# Autodesk Inventor assembly: serwo_v2
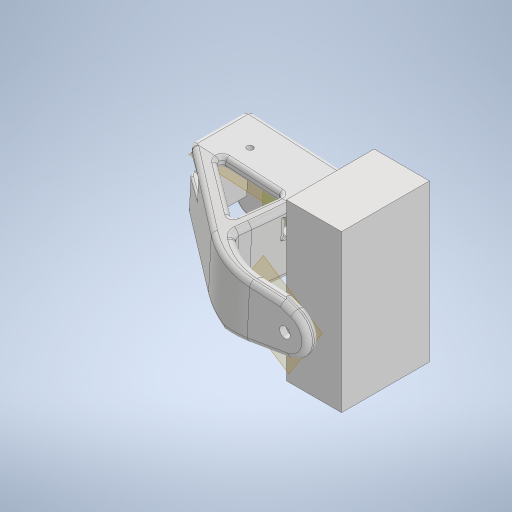
[picture p0: Inventor's stored thumbnail of the model, 512x512]
Saved by Autodesk Inventor 2023 (Build 270158000, 158)
## iProperties
Created: 2024-06-29
Part Number: serwo_v2
Document SubType Name: Assembly
Designer: kamil
Author: kamil
## Documents named in this file (4)
- C:\Users\kamil\Documents\PROJECTS - repos\Robal-2.0\mechanics\serwo_v2.iam
- C:\Users\kamil\Documents\PROJECTS - repos\Robal-2.0\mechanics\uchwyt_serwa_czlon0_pre.ipt
- C:\Users\kamil\Documents\PROJECTS - repos\Robal-2.0\mechanics\Standard-Servo.ipt
- C:\Users\kamil\Documents\PROJECTS - repos\Robal-2.0\mechanics\czlon2_pre.ipt
## Components (3 placed, 3 different names)
1. uchwyt_serwa_czlon0_pre:1 — Zestawiające:1, Zestawiające:2, Zestawiające:3
2. Standard-Servo:1 — Zestawiające:1, Zestawiające:2, Zestawiające:3, Zestawiające:4, Zestawiające:5
3. czlon2_pre:1 — Zestawiające:4, Zestawiające:5
## Relationships (5: Mate 5)
- Zestawiające:1 [Mate]: uchwyt_serwa_czlon0_pre:1 ↔ Standard-Servo:1
- Zestawiające:2 [Mate] (1 mm): uchwyt_serwa_czlon0_pre:1 ↔ Standard-Servo:1
- Zestawiające:3 [Mate] (1 mm): uchwyt_serwa_czlon0_pre:1 ↔ Standard-Servo:1
- Zestawiające:4 [Mate] (2.1 mm): Standard-Servo:1 ↔ czlon2_pre:1
- Zestawiające:5 [Mate]: Standard-Servo:1 ↔ czlon2_pre:1
